# Autodesk Inventor assembly: shoulder_roll_actuator
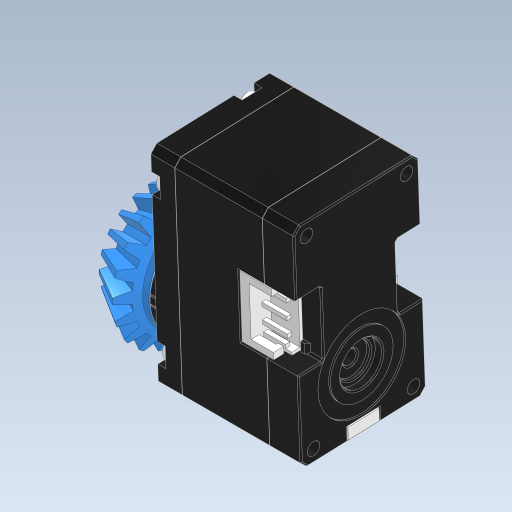
[picture p0: Inventor's stored thumbnail of the model, 512x512]
Saved by Autodesk Inventor 2024 (Build 280153000, 153)
## iProperties
Created: 2023-09-03
Part Number: shoulder_roll_actuator
Document SubType Name: Assembly
Designer: michi
Author: michi
## Documents named in this file (4)
- C:\Users\michi\OneDrive - Kyoto University\lab\6_SHINOBI\FUHGA4\Design_Mechanism\5_birdeye\birdeye_shoulderUnit\birdeye_shoulderUnit_actuator.iam
- C:\Users\michi\OneDrive - Kyoto University\lab\6_SHINOBI\FUHGA4\Design_Mechanism\5_birdeye\birdeye_shoulderUnit\birdeye_shoulderUnit_gear-small.ipt
- C:\Users\michi\OneDrive - Kyoto University\lab\6_SHINOBI\FUHGA4\Design_Mechanism\0_devices\Dynamixel\X330\XL,XC-330.iam
- C:\Users\michi\OneDrive - Kyoto University\lab\6_SHINOBI\FUHGA4\Design_Mechanism\5_birdeye\birdeye_shoulderUnit\_SPA-SUS-D1.6-6.ipt
## Components (6 placed, 3 different names)
1. birdeye_shoulderUnit_gear-small:1 — 回転:1, メイト:1, メイト:2
2. XL,XC-330:1 [sub-assembly] — 回転:1, メイト:1, メイト:3
3. _SPA-SUS-D1.6-6:1 — メイト:2, メイト:3
4. _SPA-SUS-D1.6-6:2
5. _SPA-SUS-D1.6-6:3
6. _SPA-SUS-D1.6-6:4
## Component patterns: (4 elements, first: _SPA-SUS-D1.6-6:1)
## Relationships (4: Mate 3, RevoluteJoint 1)
- 回転:1 [RevoluteJoint]: birdeye_shoulderUnit_gear-small:1 ↔ XL,XC-330:1
- メイト:1 [Mate]: birdeye_shoulderUnit_gear-small:1 ↔ XL,XC-330:1
- メイト:2 [Mate]: birdeye_shoulderUnit_gear-small:1 ↔ _SPA-SUS-D1.6-6:1
- メイト:3 [Mate] (-2.5 mm): XL,XC-330:1 ↔ _SPA-SUS-D1.6-6:1
